# Autodesk Inventor assembly: Ensamble
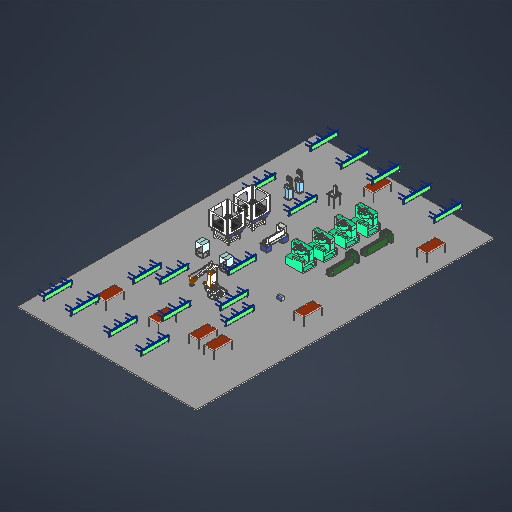
[picture p0: Inventor's stored thumbnail of the model, 512x512]
Saved by Autodesk Inventor 2026.2 (Build 302298000, 298)
## iProperties
Created: 2025-11-25
Part Number: Ensamble
Document SubType Name: Assembly
Designer: USUARIO
Author: USUARIO
## Documents named in this file (14)
- F:\UNAL\14. SEMESTRE\AUTOMATIZACIÓN DE PROCESOS DE MANUFACTURA\GitHub\Los4Automaticos\CAD\InventorProyecto\Ensamble.iam
- F:\UNAL\14. SEMESTRE\AUTOMATIZACIÓN DE PROCESOS DE MANUFACTURA\GitHub\Los4Automaticos\CAD\InventorProyecto\Floor.ipt
- F:\UNAL\14. SEMESTRE\AUTOMATIZACIÓN DE PROCESOS DE MANUFACTURA\GitHub\Los4Automaticos\CAD\InventorProyecto\Talladora.ipt
- F:\UNAL\14. SEMESTRE\AUTOMATIZACIÓN DE PROCESOS DE MANUFACTURA\GitHub\Los4Automaticos\CAD\InventorProyecto\Torno1.ipt
- F:\UNAL\14. SEMESTRE\AUTOMATIZACIÓN DE PROCESOS DE MANUFACTURA\GitHub\Los4Automaticos\CAD\InventorProyecto\Torno2.ipt
- F:\UNAL\14. SEMESTRE\AUTOMATIZACIÓN DE PROCESOS DE MANUFACTURA\GitHub\Los4Automaticos\CAD\InventorProyecto\FresadoraGrande.ipt
- F:\UNAL\14. SEMESTRE\AUTOMATIZACIÓN DE PROCESOS DE MANUFACTURA\GitHub\Los4Automaticos\CAD\InventorProyecto\FresadoraPequeña.ipt
- F:\UNAL\14. SEMESTRE\AUTOMATIZACIÓN DE PROCESOS DE MANUFACTURA\GitHub\Los4Automaticos\CAD\InventorProyecto\Taladro.ipt
- F:\UNAL\14. SEMESTRE\AUTOMATIZACIÓN DE PROCESOS DE MANUFACTURA\GitHub\Los4Automaticos\CAD\InventorProyecto\Verificadora.ipt
- F:\UNAL\14. SEMESTRE\AUTOMATIZACIÓN DE PROCESOS DE MANUFACTURA\GitHub\Los4Automaticos\CAD\InventorProyecto\CabinaPintura.ipt
- F:\UNAL\14. SEMESTRE\AUTOMATIZACIÓN DE PROCESOS DE MANUFACTURA\GitHub\Los4Automaticos\CAD\InventorProyecto\Robot.ipt
- F:\UNAL\14. SEMESTRE\AUTOMATIZACIÓN DE PROCESOS DE MANUFACTURA\GitHub\Los4Automaticos\CAD\InventorProyecto\Gripper.ipt
- F:\UNAL\14. SEMESTRE\AUTOMATIZACIÓN DE PROCESOS DE MANUFACTURA\GitHub\Los4Automaticos\CAD\InventorProyecto\MesaEnsamble.iam
- F:\UNAL\14. SEMESTRE\AUTOMATIZACIÓN DE PROCESOS DE MANUFACTURA\GitHub\Los4Automaticos\CAD\InventorProyecto\Banda.iam
## Components (42 placed, 13 different names)
1. Floor:1 — Coincidencia:7, Coincidencia:8, Coincidencia:9, Coincidencia:10, Coincidencia:11, Coincidencia:12, Coincidencia:13, Coincidencia:14, Coincidencia:15, Coincidencia:16, Coincidencia:24, Coincidencia:25, Coincidencia:26, Coincidencia:27, Coincidencia:28, Coincidencia:29, Coincidencia:30, Coincidencia:31, Coincidencia:32, Coincidencia:33, Coincidencia:34, Coincidencia:35, Coincidencia:36
2. Torno1:1 — Coincidencia:14
3. Torno2:1 — Coincidencia:25
4. Torno2:2 — Coincidencia:24
5. FresadoraGrande:1 — Coincidencia:16
6. FresadoraGrande:2 — Coincidencia:15
7. FresadoraPequeña:1 — Coincidencia:12
8. FresadoraPequeña:2 — Coincidencia:13
9. Taladro:1 — Coincidencia:11
10. Verificadora:1 — Coincidencia:8
11. Verificadora:2 — Coincidencia:7
12. CabinaPintura:1 — Coincidencia:10
13. Robot:1 — Coincidencia:9, Insertar:1
14. Gripper:1 — Insertar:1
15. Talladora:1 — Coincidencia:29
16. Talladora:2 — Coincidencia:28
17. Talladora:3 — Coincidencia:27
18. Talladora:4 — Coincidencia:26
19. MesaEnsamble:1 [sub-assembly] — Coincidencia:35
20. MesaEnsamble:2 [sub-assembly] — Coincidencia:36
21. MesaEnsamble:3 [sub-assembly] — Coincidencia:34
22. MesaEnsamble:4 [sub-assembly] — Coincidencia:33
23. MesaEnsamble:5 [sub-assembly] — Coincidencia:32
24. MesaEnsamble:6 [sub-assembly] — Coincidencia:31
25. MesaEnsamble:7 [sub-assembly] — Coincidencia:30
26. Banda:1 [sub-assembly]
27. Banda:2 [sub-assembly]
28. Banda:3 [sub-assembly]
29. Banda:4 [sub-assembly]
30. Banda:5 [sub-assembly]
31. Banda:6 [sub-assembly]
32. Banda:7 [sub-assembly]
33. Banda:8 [sub-assembly]
34. Banda:9 [sub-assembly]
35. Banda:10 [sub-assembly]
36. Banda:11 [sub-assembly]
37. Banda:12 [sub-assembly]
38. Banda:13 [sub-assembly]
39. Banda:14 [sub-assembly]
40. Banda:15 [sub-assembly]
41. Banda:16 [sub-assembly]
42. Banda:17 [sub-assembly]
## Relationships (24: Mate 23, Insert 1)
- Coincidencia:7 [Mate]: Floor:1 ↔ Verificadora:2
- Coincidencia:8 [Mate]: Floor:1 ↔ Verificadora:1
- Coincidencia:9 [Mate]: Floor:1 ↔ Robot:1
- Coincidencia:10 [Mate]: Floor:1 ↔ CabinaPintura:1
- Coincidencia:11 [Mate]: Floor:1 ↔ Taladro:1
- Coincidencia:12 [Mate]: Floor:1 ↔ FresadoraPequeña:1
- Coincidencia:13 [Mate]: Floor:1 ↔ FresadoraPequeña:2
- Coincidencia:14 [Mate]: Floor:1 ↔ Torno1:1
- Coincidencia:15 [Mate]: Floor:1 ↔ FresadoraGrande:2
- Coincidencia:16 [Mate]: Floor:1 ↔ FresadoraGrande:1
- Insertar:1: Robot:1 ↔ Gripper:1
- Coincidencia:24 [Mate]: Floor:1 ↔ Torno2:2
- Coincidencia:25 [Mate]: Floor:1 ↔ Torno2:1
- Coincidencia:26 [Mate]: Floor:1 ↔ Talladora:4
- Coincidencia:27 [Mate]: Floor:1 ↔ Talladora:3
- Coincidencia:28 [Mate]: Floor:1 ↔ Talladora:2
- Coincidencia:29 [Mate]: Floor:1 ↔ Talladora:1
- Coincidencia:30 [Mate]: Floor:1 ↔ MesaEnsamble:7
- Coincidencia:31 [Mate]: Floor:1 ↔ MesaEnsamble:6
- Coincidencia:32 [Mate]: Floor:1 ↔ MesaEnsamble:5
- Coincidencia:33 [Mate]: Floor:1 ↔ MesaEnsamble:4
- Coincidencia:34 [Mate]: Floor:1 ↔ MesaEnsamble:3
- Coincidencia:35 [Mate]: Floor:1 ↔ MesaEnsamble:1
- Coincidencia:36 [Mate]: Floor:1 ↔ MesaEnsamble:2
